# Autodesk Inventor assembly: Chessboard Design
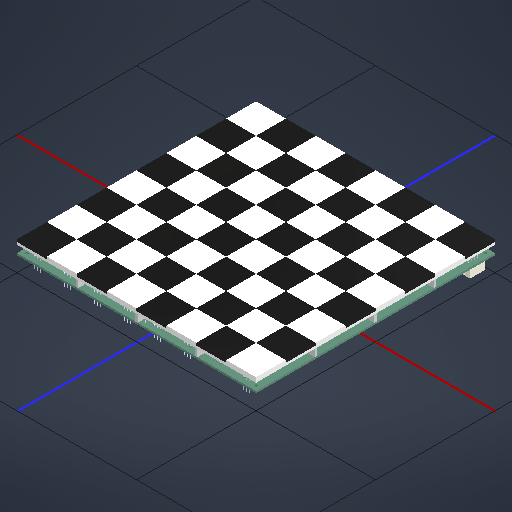
[picture p0: Inventor's stored thumbnail of the model, 512x512]
Saved by Autodesk Inventor 2026 (Build 300175000, 175)
## iProperties
Created: 2025-04-19
Part Number: Chessboard Design
Document SubType Name: Assembly
Designer: ckyiu
Author: ckyiu
## Documents named in this file (4)
- C:\Users\ckyiu\Documents\Projects\Chessboard-Design\Chessboard Design.iam
- C:\Users\ckyiu\Documents\Projects\Chessboard-Design\Assemblies\Chessboard Top.iam
- C:\Users\ckyiu\Documents\Projects\Chessboard-Design\Assemblies\PCBs\Chessboard Hardware Model.iam
- C:\Users\ckyiu\Documents\Projects\Chessboard-Design\Parts\Square Holder Support.ipt
## Components (3 placed, 3 different names)
1. Chessboard Top:1 [sub-assembly] — Flush:1, Flush:2, Mate:2
2. Chessboard Hardware Model:1 [sub-assembly] — Flush:1, Flush:2, Flush:3, Flush:4, Mate:1
3. Square Holder Support:1 — Flush:3, Flush:4, Mate:1, Mate:2
## Relationships (6: Flush 4, Mate 2)
- Flush:1: Chessboard Top:1 ↔ Chessboard Hardware Model:1
- Flush:2: Chessboard Top:1 ↔ Chessboard Hardware Model:1
- Flush:3: Chessboard Hardware Model:1 ↔ Square Holder Support:1
- Flush:4: Chessboard Hardware Model:1 ↔ Square Holder Support:1
- Mate:1: Chessboard Hardware Model:1 ↔ Square Holder Support:1
- Mate:2: Chessboard Top:1 ↔ Square Holder Support:1
